# Autodesk Inventor assembly: ASY ДМФ 040 кольцо под шпильки КОРМА
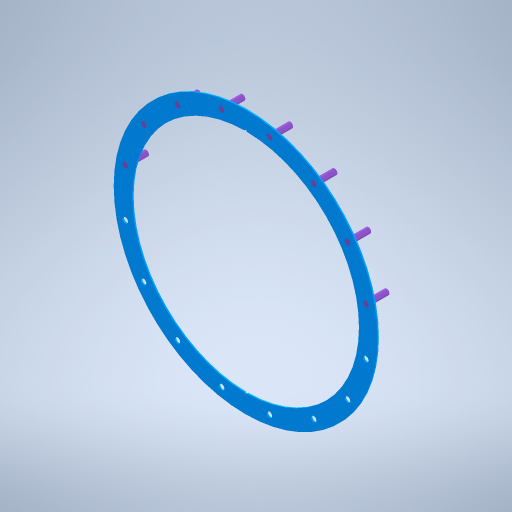
[picture p0: Inventor's stored thumbnail of the model, 512x512]
Saved by Autodesk Inventor 2024.2 (Build 282272000, 272)
## iProperties
Created: 2024-05-08
Part Number: ASY ДМФ 040 кольцо под шпильки КОРМА
Document SubType Name: Assembly
Designer: pokla
Stock Number: ДМФ 040 кольцо под шпильки КОРМА
Author: pokla
## Documents named in this file (4)
- C:\Users\user\YandexDisk\домашниий пк\Inventor\DMF-Disk-Micro-Filter\ASY ДМФ 040 кольцо под шпильки КОРМА.iam
- C:\Users\user\YandexDisk\домашниий пк\Inventor\DMF-Disk-Micro-Filter\ДМФ 041 кольцо под шпильки КОРМА.ipt
- C:\Users\user\YandexDisk\домашниий пк\Inventor\DMF-Disk-Micro-Filter\ДМФ 000 размеры.ipt
- C:\Users\user\YandexDisk\домашниий пк\Inventor\DMF-Disk-Micro-Filter\ДМФ 043 шпилька 2.ipt
## Components (9 placed, 2 different names)
1. ДМС 011 кольцо под шпильки корма:1 — Rigid:2
2. ДМФ 043 шпилька 2:1 — Rigid:2
3. ДМФ 043 шпилька 2:2
4. ДМФ 043 шпилька 2:3
5. ДМФ 043 шпилька 2:4
6. ДМФ 043 шпилька 2:5
7. ДМФ 043 шпилька 2:6
8. ДМФ 043 шпилька 2:7
9. ДМФ 043 шпилька 2:8
## Component patterns: (8 elements, first: ДМФ 043 шпилька 2:1)
## Relationships (1: WeldJoint 1)
- Rigid:2 [WeldJoint]: ДМС 011 кольцо под шпильки корма:1 ↔ ДМФ 043 шпилька 2:1
